# Autodesk Inventor assembly: Zyklon
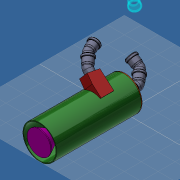
[picture p0: Inventor's stored thumbnail of the model, 180x180]
Saved by Autodesk Inventor 2019 (Build 230136000, 136)
## iProperties
Created: 2020-07-30
Part Number: Zyklon
Material: Generisch
Document SubType Name: Assembly
Designer: Stefan
Mass: 3018.8 g
Surface Area: 10924.8 cm^2
Volume: 3018.8 cm^3
Density: 1 g/cm^3
Author: Stefan
## Documents named in this file (8)
- C:\Users\User\OneDrive\Dokumente\Inventor\Absauganlage\Zyklon.iam
- C:\Users\User\OneDrive\Dokumente\Inventor\Absauganlage\Zyklon_Basis.ipt
- C:\Users\User\OneDrive\Dokumente\Inventor\Absauganlage\Zyklon_Deckel.ipt
- C:\Users\User\OneDrive\Dokumente\Inventor\Absauganlage\Zyklon_Flansch.ipt
- C:\Users\User\OneDrive\Dokumente\Inventor\Absauganlage\Zyklon_Konus.ipt
- C:\Users\User\OneDrive\Dokumente\Inventor\Absauganlage\Zyklon_Lufteinlass.ipt
- C:\Users\User\OneDrive\Dokumente\Inventor\Absauganlage\Zyklon_Stutzen.ipt
- C:\Users\User\OneDrive\Dokumente\Inventor\Absauganlage\Import\HT_Rohr\HT-50-500mm-3-69.iam
## Components (7 placed, 7 different names)
1. Zyklon_Basis:1 — Passend:1, Passend:2, Passend:3, Passend:4
2. Zyklon_Deckel:1 — Passend:3, Passend:4, Passend:5, Passend:6, Passend:7, Fluchtend:3
3. Zyklon_Flansch:1 — Passend:5, Passend:6
4. Zyklon_Konus:1 — Passend:9, Passend:10, Passend:12
5. Zyklon_Lufteinlass:1 — Passend:11, Passend:12
6. Zyklon_Stutzen:1 — Passend:1, Passend:2
7. HT-50-500mm-3-69:1 [sub-assembly] — Passend:7, Passend:9, Passend:10, Passend:11, Fluchtend:3
## Relationships (12: Mate 11, Flush 1)
- Passend:1 [Mate]: Zyklon_Basis:1 ↔ Zyklon_Stutzen:1
- Passend:2 [Mate]: Zyklon_Basis:1 ↔ Zyklon_Stutzen:1
- Passend:3 [Mate]: Zyklon_Basis:1 ↔ Zyklon_Deckel:1
- Passend:4 [Mate]: Zyklon_Basis:1 ↔ Zyklon_Deckel:1
- Passend:5 [Mate]: Zyklon_Deckel:1 ↔ Zyklon_Flansch:1
- Passend:6 [Mate]: Zyklon_Deckel:1 ↔ Zyklon_Flansch:1
- Passend:7 [Mate]: Zyklon_Deckel:1 ↔ HT-50-500mm-3-69:1
- Passend:9 [Mate]: Zyklon_Konus:1 ↔ HT-50-500mm-3-69:1
- Passend:10 [Mate]: Zyklon_Konus:1 ↔ HT-50-500mm-3-69:1
- Passend:11 [Mate]: Zyklon_Lufteinlass:1 ↔ HT-50-500mm-3-69:1
- Passend:12 [Mate]: Zyklon_Konus:1 ↔ Zyklon_Lufteinlass:1
- Fluchtend:3 [Flush] (-55 mm): Zyklon_Deckel:1 ↔ HT-50-500mm-3-69:1
